# Autodesk Inventor assembly: Baugruppe1
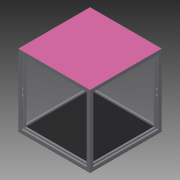
[picture p0: Inventor's stored thumbnail of the model, 180x180]
Saved by Autodesk Inventor 2018.2 (Build 222227000, 227)
## iProperties
Created: 2019-09-20
Part Number: Baugruppe1
Material: Generisch
Document SubType Name: Assembly
Designer: Lolob
Author: Lolob
## Documents named in this file (11)
- C:\Users\Lolob\Documents\Dipl\Smartcube_Construction\Version_3\Baugruppe1.iam
- C:\Users\Lolob\Documents\Dipl\Smartcube_Construction\Version_2\PV_Modul.ipt
- C:\Users\Lolob\Documents\Dipl\Smartcube_Construction\Version_2\PV_Modul_CPY.ipt
- C:\Users\Lolob\Documents\Dipl\Smartcube_Construction\Version_2\PV_Ramen_CPY_3.ipt
- C:\Users\Lolob\Documents\Dipl\Smartcube_Construction\Version_2\PV_Modul_CPY_3.ipt
- C:\Users\Lolob\Documents\Dipl\Smartcube_Construction\Version_2\PV_Modul_CPY_3_3.ipt
- C:\Users\Lolob\Documents\Dipl\Smartcube_Construction\Version_3\Boden.ipt
- C:\Users\Lolob\Documents\Dipl\Smartcube_Construction\Version_2\PV_Ramen_CPY_3_21.ipt
- C:\Users\Lolob\Documents\Dipl\Smartcube_Construction\Version_2\PV_Ramen_CPY_3_21_2.ipt
- C:\Users\Lolob\Documents\Dipl\Smartcube_Construction\Version_2\PV_Ramen_CPY_3_21_21.ipt
- C:\Users\Lolob\Documents\Dipl\Smartcube_Construction\Version_3\Boden_2.ipt
## Components (10 placed, 10 different names)
1. Boden:1 — Starr:5, Starr:6, Starr:7
2. PV_Modul:1
3. PV_Modul_CPY:1
4. PV_Ramen_CPY_3:1 — Starr:4, Passend:5, Passend:6, Passend:10, Passend:11, Fluchtend:1, Starr:8
5. PV_Modul_CPY_3:1 — Starr:4
6. PV_Modul_CPY_3_3:1
7. PV_Ramen_CPY_3_21:1 — Passend:12, Passend:13, Fluchtend:2, Passend:14, Passend:15, Starr:6
8. PV_Ramen_CPY_3_21_2:1 — Passend:16, Passend:17, Passend:18, Passend:19, Fluchtend:3, Starr:7
9. PV_Ramen_CPY_3_21_21:1 — Passend:20, Passend:21, Passend:22, Passend:23, Fluchtend:4, Starr:5
10. Boden_2:1 — Starr:8
## Relationships (25: Mate 16, WeldJoint 5, Flush 4)
- Starr:4 [WeldJoint]: PV_Ramen_CPY_3:1 ↔ PV_Modul_CPY_3:1
- Passend:5 [Mate]: PV_Ramen_CPY_3:1
- Passend:6 [Mate]: PV_Ramen_CPY_3:1
- Passend:10 [Mate]: PV_Ramen_CPY_3:1
- Passend:11 [Mate]: PV_Ramen_CPY_3:1
- Fluchtend:1 [Flush]: PV_Ramen_CPY_3:1
- Passend:12 [Mate]: PV_Ramen_CPY_3_21:1
- Passend:13 [Mate]: PV_Ramen_CPY_3_21:1
- Fluchtend:2 [Flush]: PV_Ramen_CPY_3_21:1
- Passend:14 [Mate]: PV_Ramen_CPY_3_21:1
- Passend:15 [Mate]: PV_Ramen_CPY_3_21:1
- Passend:16 [Mate]: PV_Ramen_CPY_3_21_2:1
- Passend:17 [Mate]: PV_Ramen_CPY_3_21_2:1
- Passend:18 [Mate]: PV_Ramen_CPY_3_21_2:1
- Passend:19 [Mate]: PV_Ramen_CPY_3_21_2:1
- Fluchtend:3 [Flush]: PV_Ramen_CPY_3_21_2:1
- Passend:20 [Mate]: PV_Ramen_CPY_3_21_21:1
- Passend:21 [Mate]: PV_Ramen_CPY_3_21_21:1
- Passend:22 [Mate]: PV_Ramen_CPY_3_21_21:1
- Passend:23 [Mate]: PV_Ramen_CPY_3_21_21:1
- Fluchtend:4 [Flush]: PV_Ramen_CPY_3_21_21:1
- Starr:5 [WeldJoint]: Boden:1 ↔ PV_Ramen_CPY_3_21_21:1
- Starr:6 [WeldJoint]: Boden:1 ↔ PV_Ramen_CPY_3_21:1
- Starr:7 [WeldJoint]: Boden:1 ↔ PV_Ramen_CPY_3_21_2:1
- Starr:8 [WeldJoint]: PV_Ramen_CPY_3:1 ↔ Boden_2:1
